# Autodesk Inventor assembly: Montagem do robô completo
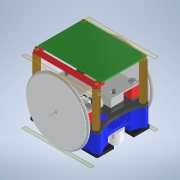
[picture p0: Inventor's stored thumbnail of the model, 180x180]
Saved by Autodesk Inventor 2021 (Build 250183000, 183)
## iProperties
Created: 2021-11-20
Part Number: Montagem do robô completo
Document SubType Name: Assembly
Designer: Matheus
Mass: 252.38 g
Surface Area: 890.07 cm^2
Volume: 110.055 cm^3
Density: 2.29323 g/cm^3
Author: Matheus
## Documents named in this file (23)
- D:\Projetos\Robo_TCC\Montagem do robô completo.iam
- D:\Projetos\Robo_TCC\Motor HP 100-1 Pololu eixo estendido.ipt
- D:\Projetos\Robo_TCC\Encoder lateral.ipt
- D:\Projetos\Robo_TCC\Disco encoder magnético.ipt
- D:\Projetos\Robo_TCC\Tampa motores.ipt
- D:\Projetos\Robo_TCC\Rolamento 6x3x2mm.ipt
- D:\Projetos\Robo_TCC\Eixo da roda.ipt
- D:\Projetos\Robo_TCC\MontagemPneuRoda.iam
- D:\Projetos\Robo_TCC\Mancal superior.ipt
- D:\Projetos\Robo_TCC\Piso dos motores.ipt
- D:\Projetos\Robo_TCC\Parafuso - M3x0,5 x 20.ipt
- C:\Users\Mathe\OneDrive\Documentos\Inventor\Content Center Files\R2021\en-US\ANSI B 18.2.4.1 M(1)\ANSI B 18.2.4.1 M - M3 x 0,5Style 1.ipt
- D:\Projetos\Robo_TCC\Suporte Ball Caster Max.ipt
- D:\Projetos\Robo_TCC\Ball Caster.ipt
- D:\Projetos\Robo_TCC\Placa de Aço.ipt
- D:\Projetos\Robo_TCC\espaçador sext. 20mm.ipt
- D:\Projetos\Robo_TCC\Plaquinha.ipt
- D:\Projetos\Robo_TCC\Suporte placa 1 lado.ipt
- D:\Projetos\Robo_TCC\Bateria.ipt
- D:\Projetos\Robo_TCC\Engrenagem\Design Accelerator\Engrenagem reta22.ipt
- D:\Projetos\Robo_TCC\Separador engrenagens.ipt
- D:\Projetos\Robo_TCC\Porca - M3 x 0,5.ipt
- D:\Projetos\Robo_TCC\Parafuso - M3x0,5 x 30.ipt
## Components (63 placed, 22 different names)
1. Piso dos motores:2 — Mate:67, Flush:8, Mate:70, Mate:71, Mate:72, Mate:73, Mate:74, Mate:75, Mate:77, Mate:82, Mate:83, Mate:87, Mate:91, Mate:92, Angle:5, Angle:6, Angle:7, Mate:95, Flush:9, Flush:10, Flush:11, Mate:98, Flush:12, Mate:99, Flush:13, Mate:100, Flush:14, Mate:101, Flush:15, Mate:116, Mate:117, Mate:118, Mate:119, Mate:120, Mate:121, Mate:145, Mate:146, Mate:147, Mate:153, Mate:155, Mate:156, Mate:170
2. Tampa motores:1 — Mate:67, Flush:8, Mate:103, Mate:105, Mate:107, Mate:138, Mate:139, Angle:12, Angle:14, Angle:15, Mate:184
3. Motor HP 100-1 Pololu eixo estendido:1 — Mate:42, Mate:43, Mate:47, Flush:4, Mate:70, Mate:71, Mate:72, Mate:182, Flush:26
4. Motor HP 100-1 Pololu eixo estendido:2 — Mate:44, Mate:45, Mate:46, Flush:3, Mate:73, Mate:74, Mate:75, Mate:180, Flush:24
5. Mancal superior:1 — Mate:77, Mate:112, Mate:113, Mate:140, Mate:141, Angle:17, Angle:18
6. Mancal superior:2 — Mate:82, Mate:114, Mate:115, Mate:142, Mate:143, Angle:13, Angle:16
7. Eixo da roda:2 — Mate:63, Mate:65, Flush:7, Mate:92, Mate:183
8. Eixo da roda:1 — Mate:61, Mate:64, Flush:6, Mate:91, Mate:181
9. Encoder lateral:1 — Mate:42, Mate:43, Angle:6
10. Encoder lateral:2 — Mate:44, Mate:45, Angle:7
11. Disco encoder magnético:1 — Mate:46, Flush:3
12. Disco encoder magnético:2 — Mate:47, Flush:4
13. Rolamento 6x3x2mm:1 — Mate:51, Mate:87, Mate:89, Mate:146
14. Rolamento 6x3x2mm:2 — Mate:57, Mate:83, Mate:85, Mate:145
15. Rolamento 6x3x2mm:3 — Mate:51, Mate:53, Mate:89, Mate:90
16. Rolamento 6x3x2mm:4 — Mate:53, Mate:61, Mate:90
17. Rolamento 6x3x2mm:5 — Mate:59, Mate:63, Mate:86
18. Rolamento 6x3x2mm:6 — Mate:57, Mate:59, Mate:85, Mate:86
19. MontagemPneuRoda:1 [sub-assembly] — Mate:64, Flush:6, Angle:4
20. MontagemPneuRoda:2 [sub-assembly] — Mate:65, Flush:7, Angle:4, Angle:5
21. Parafuso - M3x0,5 x 20:1 — Mate:99, Flush:13, Mate:110, Mate:140, Mate:192
22. Parafuso - M3x0,5 x 20:2 — Mate:98, Flush:12, Mate:111, Mate:141, Mate:185, Mate:188
23. Parafuso - M3x0,5 x 20:3 — Flush:11, Mate:102, Mate:147
24. Parafuso - M3x0,5 x 20:4 — Mate:101, Flush:15, Mate:108, Mate:143, Mate:186, Mate:193
25. Parafuso - M3x0,5 x 20:5 — Mate:100, Flush:14, Mate:109, Mate:142, Mate:190
26. Parafuso - M3x0,5 x 20:6 — Mate:95, Flush:9, Mate:104, Mate:139
27. Parafuso - M3x0,5 x 20:7 — Flush:10, Mate:106, Mate:138
28. Hex Nut Metric M3 x 0,5:2 — Mate:102, Mate:103, Angle:15
29. Hex Nut Metric M3 x 0,5:3 — Mate:106, Mate:107, Angle:12
30. Hex Nut Metric M3 x 0,5:4 — Mate:109, Mate:115, Angle:13
31. Hex Nut Metric M3 x 0,5:5 — Mate:108, Mate:114, Angle:16
32. Hex Nut Metric M3 x 0,5:6 — Mate:104, Mate:105, Angle:14
33. Hex Nut Metric M3 x 0,5:7 — Mate:110, Mate:113, Angle:17
34. Hex Nut Metric M3 x 0,5:8 — Mate:111, Mate:112, Angle:18
35. Suporte Ball Caster Max:1 — Mate:116, Mate:117, Mate:118, Mate:124, Mate:125, Mate:126, Mate:133, Angle:10, Angle:11
36. Suporte Ball Caster Max:2 — Mate:119, Mate:120, Mate:121, Mate:122, Mate:123, Mate:137, Mate:144, Mate:134, Mate:163, Angle:8, Angle:9
37. Ball Caster:1 — Mate:122, Mate:123, Mate:144
38. Ball Caster:2 — Mate:124, Mate:125, Mate:126
39. Placa de Aço:1 — Mate:133, Mate:134, Mate:137, Mate:160, Mate:161, Mate:162, Mate:163, Mate:195, Flush:28, Mate:196, Mate:197, Mate:198, Flush:29, Mate:199, Flush:30
40. espaçador sext. 20mm:1 — Mate:156, Angle:10, Mate:168, Mate:169, Flush:22
41. espaçador sext. 20mm:3 — Mate:153, Angle:9, Mate:166, Mate:167, Flush:21
42. espaçador sext. 20mm:4 — Mate:155, Mate:164, Mate:165, Flush:20, Angle:8
43. Plaquinha:1 — Mate:177, Mate:178, Mate:179
44. Suporte placa 1 lado:1 — Mate:174, Mate:175, Mate:176, Mate:177, Mate:178, Mate:179
45. Bateria:1 — Mate:160, Mate:161, Mate:162
46. espaçador sext. 20mm:5 — Mate:172, Mate:173, Flush:23, Mate:176
47. espaçador sext. 20mm:6 — Mate:170, Angle:11, Mate:172, Mate:173, Flush:23
48. espaçador sext. 20mm:7 — Mate:168, Mate:169, Flush:22
49. espaçador sext. 20mm:8 — Mate:166, Mate:167, Flush:21
50. espaçador sext. 20mm:9 — Mate:164, Mate:165, Flush:20, Mate:174, Mate:175
51. Engrenagem reta2:1 — Mate:180, Flush:24, Flush:25
52. Engrenagem reta2:2 — Mate:182, Flush:26, Flush:27
53. Engrenagem reta2:3 — Mate:183, Flush:27
54. Engrenagem reta2:4 — Mate:181, Flush:25
55. Separador engrenagens:1 — Mate:184, Mate:185, Mate:186, Mate:187, Mate:189, Mate:191, Mate:194
56. Porca - M3 x 0,5:1 — Mate:189, Mate:190
57. Porca - M3 x 0,5:2 — Mate:191, Mate:192
58. Porca - M3 x 0,5:3 — Mate:193, Mate:194
59. Porca - M3 x 0,5:4 — Mate:187, Mate:188
60. Parafuso - M3x0,5 x 30:1 — Mate:198, Flush:29
61. Parafuso - M3x0,5 x 30:2 — Mate:195, Flush:28
62. Parafuso - M3x0,5 x 30:3 — Mate:196, Mate:197
63. Parafuso - M3x0,5 x 30:4 — Mate:199, Flush:30
## Relationships (154: Mate 116, Flush 23, Angle 15)
- Mate:42: Motor HP 100-1 Pololu eixo estendido:1 ↔ Encoder lateral:1
- Mate:43: Motor HP 100-1 Pololu eixo estendido:1 ↔ Encoder lateral:1
- Mate:44: Motor HP 100-1 Pololu eixo estendido:2 ↔ Encoder lateral:2
- Mate:45: Motor HP 100-1 Pololu eixo estendido:2 ↔ Encoder lateral:2
- Mate:46: Motor HP 100-1 Pololu eixo estendido:2 ↔ Disco encoder magnético:1
- Flush:3: Motor HP 100-1 Pololu eixo estendido:2 ↔ Disco encoder magnético:1
- Mate:47: Motor HP 100-1 Pololu eixo estendido:1 ↔ Disco encoder magnético:2
- Flush:4: Motor HP 100-1 Pololu eixo estendido:1 ↔ Disco encoder magnético:2
- Mate:51: Rolamento 6x3x2mm:1 ↔ Rolamento 6x3x2mm:3
- Mate:53: Rolamento 6x3x2mm:3 ↔ Rolamento 6x3x2mm:4
- Mate:57: Rolamento 6x3x2mm:2 ↔ Rolamento 6x3x2mm:6
- Mate:59: Rolamento 6x3x2mm:5 ↔ Rolamento 6x3x2mm:6
- Mate:61 (-1 mm): Eixo da roda:1 ↔ Rolamento 6x3x2mm:4
- Mate:63 (-1 mm): Eixo da roda:2 ↔ Rolamento 6x3x2mm:5
- Mate:64: Eixo da roda:1 ↔ MontagemPneuRoda:1
- Flush:6: Eixo da roda:1 ↔ MontagemPneuRoda:1
- Mate:65: Eixo da roda:2 ↔ MontagemPneuRoda:2
- Flush:7: Eixo da roda:2 ↔ MontagemPneuRoda:2
- Angle:4 (0 deg): MontagemPneuRoda:1 ↔ MontagemPneuRoda:2
- Mate:67: Piso dos motores:2 ↔ Tampa motores:1
- Flush:8: Piso dos motores:2 ↔ Tampa motores:1
- Mate:70: Piso dos motores:2 ↔ Motor HP 100-1 Pololu eixo estendido:1
- Mate:71: Piso dos motores:2 ↔ Motor HP 100-1 Pololu eixo estendido:1
- Mate:72: Piso dos motores:2 ↔ Motor HP 100-1 Pololu eixo estendido:1
- Mate:73: Piso dos motores:2 ↔ Motor HP 100-1 Pololu eixo estendido:2
- Mate:74: Piso dos motores:2 ↔ Motor HP 100-1 Pololu eixo estendido:2
- Mate:75: Piso dos motores:2 ↔ Motor HP 100-1 Pololu eixo estendido:2
- Mate:77: Piso dos motores:2 ↔ Mancal superior:1
- Mate:82: Piso dos motores:2 ↔ Mancal superior:2
- Mate:83: Piso dos motores:2 ↔ Rolamento 6x3x2mm:2
- Mate:85: Rolamento 6x3x2mm:2 ↔ Rolamento 6x3x2mm:6
- Mate:86: Rolamento 6x3x2mm:5 ↔ Rolamento 6x3x2mm:6
- Mate:87: Piso dos motores:2 ↔ Rolamento 6x3x2mm:1
- Mate:89: Rolamento 6x3x2mm:1 ↔ Rolamento 6x3x2mm:3
- Mate:90: Rolamento 6x3x2mm:3 ↔ Rolamento 6x3x2mm:4
- Mate:91: Piso dos motores:2 ↔ Eixo da roda:1
- Mate:92: Piso dos motores:2 ↔ Eixo da roda:2
- Angle:5 (0 deg): Piso dos motores:2 ↔ MontagemPneuRoda:2
- Angle:6 (180 deg): Piso dos motores:2 ↔ Encoder lateral:1
- Angle:7 (180 deg): Piso dos motores:2 ↔ Encoder lateral:2
- Mate:95: Piso dos motores:2 ↔ Parafuso - M3x0,5 x 20:6
- Flush:9: Piso dos motores:2 ↔ Parafuso - M3x0,5 x 20:6
- Flush:10: Piso dos motores:2 ↔ Parafuso - M3x0,5 x 20:7
- Flush:11: Piso dos motores:2 ↔ Parafuso - M3x0,5 x 20:3
- Mate:98: Piso dos motores:2 ↔ Parafuso - M3x0,5 x 20:2
- Flush:12: Piso dos motores:2 ↔ Parafuso - M3x0,5 x 20:2
- Mate:99: Piso dos motores:2 ↔ Parafuso - M3x0,5 x 20:1
- Flush:13: Piso dos motores:2 ↔ Parafuso - M3x0,5 x 20:1
- Mate:100: Piso dos motores:2 ↔ Parafuso - M3x0,5 x 20:5
- Flush:14: Piso dos motores:2 ↔ Parafuso - M3x0,5 x 20:5
- Mate:101: Piso dos motores:2 ↔ Parafuso - M3x0,5 x 20:4
- Flush:15: Piso dos motores:2 ↔ Parafuso - M3x0,5 x 20:4
- Mate:102: Parafuso - M3x0,5 x 20:3 ↔ Hex Nut Metric M3 x 0,5:2
- Mate:103: Tampa motores:1 ↔ Hex Nut Metric M3 x 0,5:2
- Mate:104: Parafuso - M3x0,5 x 20:6 ↔ Hex Nut Metric M3 x 0,5:6
- Mate:105: Tampa motores:1 ↔ Hex Nut Metric M3 x 0,5:6
- Mate:106: Parafuso - M3x0,5 x 20:7 ↔ Hex Nut Metric M3 x 0,5:3
- Mate:107: Tampa motores:1 ↔ Hex Nut Metric M3 x 0,5:3
- Mate:108: Parafuso - M3x0,5 x 20:4 ↔ Hex Nut Metric M3 x 0,5:5
- Mate:109: Parafuso - M3x0,5 x 20:5 ↔ Hex Nut Metric M3 x 0,5:4
- Mate:110: Parafuso - M3x0,5 x 20:1 ↔ Hex Nut Metric M3 x 0,5:7
- Mate:111: Parafuso - M3x0,5 x 20:2 ↔ Hex Nut Metric M3 x 0,5:8
- Mate:112: Mancal superior:1 ↔ Hex Nut Metric M3 x 0,5:8
- Mate:113: Mancal superior:1 ↔ Hex Nut Metric M3 x 0,5:7
- Mate:114: Mancal superior:2 ↔ Hex Nut Metric M3 x 0,5:5
- Mate:115: Mancal superior:2 ↔ Hex Nut Metric M3 x 0,5:4
- Mate:116: Piso dos motores:2 ↔ Suporte Ball Caster Max:1
- Mate:117: Piso dos motores:2 ↔ Suporte Ball Caster Max:1
- Mate:118: Piso dos motores:2 ↔ Suporte Ball Caster Max:1
- Mate:119: Piso dos motores:2 ↔ Suporte Ball Caster Max:2
- Mate:120: Piso dos motores:2 ↔ Suporte Ball Caster Max:2
- Mate:121: Piso dos motores:2 ↔ Suporte Ball Caster Max:2
- Mate:122: Suporte Ball Caster Max:2 ↔ Ball Caster:1
- Mate:123: Suporte Ball Caster Max:2 ↔ Ball Caster:1
- Mate:124: Suporte Ball Caster Max:1 ↔ Ball Caster:2
- Mate:125: Suporte Ball Caster Max:1 ↔ Ball Caster:2
- Mate:126: Suporte Ball Caster Max:1 ↔ Ball Caster:2
- Mate:133: Suporte Ball Caster Max:1 ↔ Placa de Aço:1
- Mate:134: Suporte Ball Caster Max:2 ↔ Placa de Aço:1
- Mate:137: Suporte Ball Caster Max:2 ↔ Placa de Aço:1
- Mate:138: Tampa motores:1 ↔ Parafuso - M3x0,5 x 20:7
- Mate:139: Tampa motores:1 ↔ Parafuso - M3x0,5 x 20:6
- Mate:140: Mancal superior:1 ↔ Parafuso - M3x0,5 x 20:1
- Mate:141: Mancal superior:1 ↔ Parafuso - M3x0,5 x 20:2
- Mate:142: Mancal superior:2 ↔ Parafuso - M3x0,5 x 20:5
- Mate:143: Mancal superior:2 ↔ Parafuso - M3x0,5 x 20:4
- Mate:144: Suporte Ball Caster Max:2 ↔ Ball Caster:1
- Mate:145: Piso dos motores:2 ↔ Rolamento 6x3x2mm:2
- Mate:146: Piso dos motores:2 ↔ Rolamento 6x3x2mm:1
- Mate:147: Piso dos motores:2 ↔ Parafuso - M3x0,5 x 20:3
- Mate:153: Piso dos motores:2 ↔ espaçador sext. 20mm:3
- Mate:155: Piso dos motores:2 ↔ espaçador sext. 20mm:4
- Mate:156: Piso dos motores:2 ↔ espaçador sext. 20mm:1
- Mate:160: Placa de Aço:1 ↔ Bateria:1
- Mate:161: Placa de Aço:1 ↔ Bateria:1
- Mate:162: Placa de Aço:1 ↔ Bateria:1
- Mate:163: Suporte Ball Caster Max:2 ↔ Placa de Aço:1
- Mate:164: espaçador sext. 20mm:4 ↔ espaçador sext. 20mm:9
- Mate:165: espaçador sext. 20mm:4 ↔ espaçador sext. 20mm:9
- Flush:20: espaçador sext. 20mm:4 ↔ espaçador sext. 20mm:9
- Angle:8 (0 deg): Suporte Ball Caster Max:2 ↔ espaçador sext. 20mm:4
- Angle:9 (0 deg): Suporte Ball Caster Max:2 ↔ espaçador sext. 20mm:3
- Mate:166: espaçador sext. 20mm:3 ↔ espaçador sext. 20mm:8
- Mate:167: espaçador sext. 20mm:3 ↔ espaçador sext. 20mm:8
- Flush:21: espaçador sext. 20mm:3 ↔ espaçador sext. 20mm:8
- Angle:10 (0 deg): Suporte Ball Caster Max:1 ↔ espaçador sext. 20mm:1
- Mate:168: espaçador sext. 20mm:1 ↔ espaçador sext. 20mm:7
- Mate:169: espaçador sext. 20mm:1 ↔ espaçador sext. 20mm:7
- Flush:22: espaçador sext. 20mm:1 ↔ espaçador sext. 20mm:7
- Mate:170: Piso dos motores:2 ↔ espaçador sext. 20mm:6
- Angle:11 (0 deg): Suporte Ball Caster Max:1 ↔ espaçador sext. 20mm:6
- Mate:172: espaçador sext. 20mm:5 ↔ espaçador sext. 20mm:6
- Mate:173: espaçador sext. 20mm:5 ↔ espaçador sext. 20mm:6
- Flush:23: espaçador sext. 20mm:5 ↔ espaçador sext. 20mm:6
- Mate:174: Suporte placa 1 lado:1 ↔ espaçador sext. 20mm:9
- Mate:175: Suporte placa 1 lado:1 ↔ espaçador sext. 20mm:9
- Mate:176: Suporte placa 1 lado:1 ↔ espaçador sext. 20mm:5
- Mate:177: Plaquinha:1 ↔ Suporte placa 1 lado:1
- Mate:178: Plaquinha:1 ↔ Suporte placa 1 lado:1
- Mate:179: Plaquinha:1 ↔ Suporte placa 1 lado:1
- Angle:12 (0 deg): Tampa motores:1 ↔ Hex Nut Metric M3 x 0,5:3
- Angle:13 (0 deg): Mancal superior:2 ↔ Hex Nut Metric M3 x 0,5:4
- Mate:180: Motor HP 100-1 Pololu eixo estendido:2 ↔ Engrenagem reta2:1
- Flush:24: Motor HP 100-1 Pololu eixo estendido:2 ↔ Engrenagem reta2:1
- Mate:181: Eixo da roda:1 ↔ Engrenagem reta2:4
- Flush:25: Engrenagem reta2:1 ↔ Engrenagem reta2:4
- Mate:182: Motor HP 100-1 Pololu eixo estendido:1 ↔ Engrenagem reta2:2
- Flush:26: Motor HP 100-1 Pololu eixo estendido:1 ↔ Engrenagem reta2:2
- Mate:183: Eixo da roda:2 ↔ Engrenagem reta2:3
- Flush:27: Engrenagem reta2:2 ↔ Engrenagem reta2:3
- Angle:14 (0 deg): Tampa motores:1 ↔ Hex Nut Metric M3 x 0,5:6
- Angle:15 (0 deg): Tampa motores:1 ↔ Hex Nut Metric M3 x 0,5:2
- Angle:16 (0 deg): Mancal superior:2 ↔ Hex Nut Metric M3 x 0,5:5
- Angle:17 (0 deg): Mancal superior:1 ↔ Hex Nut Metric M3 x 0,5:7
- Angle:18 (0 deg): Mancal superior:1 ↔ Hex Nut Metric M3 x 0,5:8
- Mate:184: Tampa motores:1 ↔ Separador engrenagens:1
- Mate:185: Parafuso - M3x0,5 x 20:2 ↔ Separador engrenagens:1
- Mate:186: Parafuso - M3x0,5 x 20:4 ↔ Separador engrenagens:1
- Mate:187: Separador engrenagens:1 ↔ Porca - M3 x 0,5:4
- Mate:188: Parafuso - M3x0,5 x 20:2 ↔ Porca - M3 x 0,5:4
- Mate:189: Separador engrenagens:1 ↔ Porca - M3 x 0,5:1
- Mate:190: Parafuso - M3x0,5 x 20:5 ↔ Porca - M3 x 0,5:1
- Mate:191: Separador engrenagens:1 ↔ Porca - M3 x 0,5:2
- Mate:192: Parafuso - M3x0,5 x 20:1 ↔ Porca - M3 x 0,5:2
- Mate:193: Parafuso - M3x0,5 x 20:4 ↔ Porca - M3 x 0,5:3
- Mate:194: Separador engrenagens:1 ↔ Porca - M3 x 0,5:3
- Mate:195: Placa de Aço:1 ↔ Parafuso - M3x0,5 x 30:2
- Flush:28: Placa de Aço:1 ↔ Parafuso - M3x0,5 x 30:2
- Mate:196: Placa de Aço:1 ↔ Parafuso - M3x0,5 x 30:3
- Mate:197: Placa de Aço:1 ↔ Parafuso - M3x0,5 x 30:3
- Mate:198: Placa de Aço:1 ↔ Parafuso - M3x0,5 x 30:1
- Flush:29: Placa de Aço:1 ↔ Parafuso - M3x0,5 x 30:1
- Mate:199: Placa de Aço:1 ↔ Parafuso - M3x0,5 x 30:4
- Flush:30: Placa de Aço:1 ↔ Parafuso - M3x0,5 x 30:4
